# Autodesk Inventor assembly: prueba3
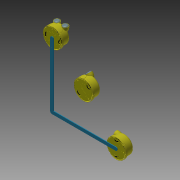
[picture p0: Inventor's stored thumbnail of the model, 180x180]
Saved by Autodesk Inventor 2015 (Build 190159000, 159)
## iProperties
Created: 2015-06-07
Part Number: prueba3
Document SubType Name: Assembly
Designer: david_000
Author: david_000
## Documents named in this file (3)
- C:\Users\david_000\Desktop\minibot-code\mechanics\prueba3.iam
- C:\Users\david_000\Desktop\minibot-code\mechanics\suelo_pruebas.ipt
- C:\Users\david_000\Desktop\minibot-code\mechanics\minibot.iam
## Components (4 placed, 2 different names)
1. suelo_pruebas:1 — Coincidencia:1, Coincidencia:2, Coincidencia:3, Ángulo:1, Ángulo:2
2. minibot:1 [sub-assembly] — Coincidencia:1, Coincidencia:2, Nivelación:1, Ángulo:1, Ángulo:3
3. minibot:2 [sub-assembly] — Tangente:1, Nivelación:2, Ángulo:3
4. minibot:3 [sub-assembly] — Coincidencia:3, Tangente:1, Nivelación:1, Nivelación:2, Ángulo:2
## Relationships (9: Mate 3, Angle 3, Flush 2, Tangent 1)
- Coincidencia:1 [Mate]: suelo_pruebas:1 ↔ minibot:1
- Coincidencia:2 [Mate]: suelo_pruebas:1 ↔ minibot:1
- Coincidencia:3 [Mate]: suelo_pruebas:1 ↔ minibot:3
- Tangente:1 (400 mm): minibot:2 ↔ minibot:3
- Nivelación:1 [Flush]: minibot:1 ↔ minibot:3
- Nivelación:2 [Flush]: minibot:2 ↔ minibot:3
- Ángulo:1 [Angle] (0 deg): suelo_pruebas:1 ↔ minibot:1
- Ángulo:2 [Angle] (0 deg): suelo_pruebas:1 ↔ minibot:3
- Ángulo:3 [Angle] (45 deg): minibot:1 ↔ minibot:2
